# Autodesk Inventor assembly: Three Jaw Chuck
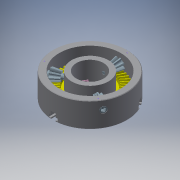
[picture p0: Inventor's stored thumbnail of the model, 180x180]
Saved by Autodesk Inventor 2016 (Build 200138000, 138)
## iProperties
Created: 2011-02-15
Part Number: Three Jaw Chuck
Document SubType Name: Assembly
Designer: nguyenducthang
Author: nguyenducthang
## Documents named in this file (8)
- C:\Users\M228854\Downloads\3 jaw final\3JawChuck1Inv\Three Jaw Chuck.iam
- C:\Users\M228854\Downloads\3 jaw final\3JawChuck1Inv\BevelB.ipt
- C:\Users\M228854\Downloads\3 jaw final\3JawChuck1Inv\BevelS.ipt
- C:\Users\M228854\Downloads\3 jaw final\3JawChuck1Inv\Base.ipt
- C:\Users\M228854\Downloads\3 jaw final\3JawChuck1Inv\Pin.ipt
- C:\Users\M228854\Downloads\3 jaw final\3JawChuck1Inv\Jaw1.ipt
- C:\Users\M228854\Downloads\3 jaw final\3JawChuck1Inv\Jaw2.ipt
- C:\Users\M228854\Downloads\3 jaw final\3JawChuck1Inv\Jaw3.ipt
## Components (11 placed, 7 different names)
1. Base:1 — Insert:1, Mate:1, Mate:2, Mate:3, Mate:4, Mate:5, Mate:6, Mate:8, Mate:10, Mate:12, Mate:13, Mate:15, Mate:16, Insert:2, Insert:3, Tangent:1, Tangent:2, Tangent:3
2. Pin:1 — Insert:1
3. BevelS:1 — Mate:1, Mate:2, Mate:9, Mate:11, Tangent:3, Rotation:1
4. BevelB:1 — Mate:3, Mate:4, Mate:7, Rotation:1, Rotation:2, Rotation:3
5. Jaw1:1 — Mate:5, Mate:6, Mate:7, Mate:14, Mate:17
6. BevelS:2 — Mate:8, Mate:9, Tangent:2, Rotation:2
7. BevelS:3 — Mate:10, Mate:11, Tangent:1, Rotation:3
8. Jaw3:1 — Mate:12, Mate:13, Mate:14
9. Jaw2:2 — Mate:15, Mate:16, Mate:17
10. Pin:2 — Insert:3
11. Pin:3 — Insert:2
## Relationships (26: Mate 17, Insert 3, Tangent 3, RelateRotation 3)
- Insert:1: Base:1 ↔ Pin:1
- Mate:1: Base:1 ↔ BevelS:1
- Mate:2: Base:1 ↔ BevelS:1
- Mate:3: Base:1 ↔ BevelB:1
- Mate:4 (0.01 mm): Base:1 ↔ BevelB:1
- Mate:5: Base:1 ↔ Jaw1:1
- Mate:6: Base:1 ↔ Jaw1:1
- Mate:7: BevelB:1 ↔ Jaw1:1
- Mate:8: Base:1 ↔ BevelS:2
- Mate:9: BevelS:1 ↔ BevelS:2
- Mate:10: Base:1 ↔ BevelS:3
- Mate:11: BevelS:1 ↔ BevelS:3
- Mate:12: Base:1 ↔ Jaw3:1
- Mate:13: Base:1 ↔ Jaw3:1
- Mate:14: Jaw1:1 ↔ Jaw3:1
- Mate:15: Base:1 ↔ Jaw2:2
- Mate:16: Base:1 ↔ Jaw2:2
- Mate:17: Jaw1:1 ↔ Jaw2:2
- Insert:2: Base:1 ↔ Pin:3
- Insert:3: Base:1 ↔ Pin:2
- Tangent:1: Base:1 ↔ BevelS:3
- Tangent:2: Base:1 ↔ BevelS:2
- Tangent:3: Base:1 ↔ BevelS:1
- Rotation:1 [RelateRotation] (3 ul): BevelS:1 ↔ BevelB:1
- Rotation:2 [RelateRotation] (3 ul): BevelB:1 ↔ BevelS:2
- Rotation:3 [RelateRotation] (3 ul): BevelB:1 ↔ BevelS:3
